# Autodesk Inventor assembly: Assembly_Opentrons_Autofocus_v1
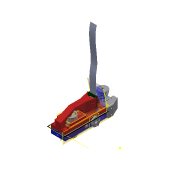
[picture p0: Inventor's stored thumbnail of the model, 180x180]
Saved by Autodesk Inventor 2019.4 (Build 234330000, 330)
## iProperties
Created: 2020-10-23
Part Number: Assembly_Opentrons_Autofocus_v1
Document SubType Name: Assembly
Designer: diederichbenedict
Author: diederichbenedict
## Documents named in this file (17)
- C:\Users\diederichbenedict\Dropbox\Dokumente\Promotion\PROJECTS\OPENTRONS\INVENTOR\Assembly_Opentrons_Autofocus_v1.iam
- C:\Users\diederichbenedict\Dropbox\Dokumente\Promotion\PROJECTS\OPENTRONS\INVENTOR\00_RasPi_Camera.ipt
- C:\Users\diederichbenedict\Dropbox\Dokumente\Promotion\PROJECTS\OPENTRONS\INVENTOR\00_IGUS_Drylin_RJ4JP-01-06.ipt
- C:\Users\diederichbenedict\Dropbox\Dokumente\Promotion\PROJECTS\OPENTRONS\INVENTOR\00_spindel_slide.ipt
- C:\Users\diederichbenedict\Dropbox\Dokumente\Promotion\PROJECTS\OPENTRONS\INVENTOR\00_objectivelens_10x.ipt
- C:\Users\diederichbenedict\Dropbox\Dokumente\Promotion\PROJECTS\OPENTRONS\INVENTOR\01_Slide_camera_x_v1.ipt
- C:\Users\diederichbenedict\Dropbox\Dokumente\Promotion\PROJECTS\OPENTRONS\INVENTOR\00_opticalpath.ipt
- C:\Users\diederichbenedict\Dropbox\Dokumente\Promotion\PROJECTS\OPENTRONS\INVENTOR\07_OPENTRONS_Autofocus_objectivemount_v0.ipt
- C:\Users\diederichbenedict\Dropbox\Dokumente\Promotion\PROJECTS\OPENTRONS\INVENTOR\00_COMAR_Mirror_10mm.ipt
- C:\Users\diederichbenedict\Dropbox\Dokumente\Promotion\PROJECTS\OPENTRONS\INVENTOR\08_Opentrons_Autofocus_flexurebaering.ipt
- C:\Users\diederichbenedict\Dropbox\Dokumente\Promotion\PROJECTS\OPENTRONS\INVENTOR\00_ESP32_Camera_only.ipt
- C:\Users\diederichbenedict\Dropbox\Dokumente\Promotion\PROJECTS\OPENTRONS\INVENTOR\00_Beampath_Autofocus _2.ipt
- C:\Users\diederichbenedict\Dropbox\Dokumente\Promotion\PROJECTS\OPENTRONS\INVENTOR\00_IR_Laserdiode.ipt
- C:\Users\diederichbenedict\Dropbox\Dokumente\Promotion\PROJECTS\OPENTRONS\INVENTOR\13_Opentrons_Autofocus_Objectivering_Laser_Cam.ipt
- C:\Users\diederichbenedict\Dropbox\Dokumente\Promotion\PROJECTS\OPENTRONS\INVENTOR\00_NEMA11.iam
- C:\Users\diederichbenedict\Dropbox\Dokumente\Promotion\PROJECTS\OPENTRONS\INVENTOR\OPENTRONS_Autofocus_NEMA_holder_tmp.ipt
- C:\Users\diederichbenedict\Dropbox\Dokumente\Promotion\PROJECTS\OPENTRONS\INVENTOR\OPENTRONS_Autofocus_spiral_Nema.ipt
## Components (16 placed, 16 different names)
1. 00_IGUS_Drylin_RJ4JP-01-06:1
2. 00_spindel_slide:1 — Insert:5
3. 01_Slide_camera_x_v1:1 — Insert:5, Mate:1, Mate:2, Flush:4, Angle:2, Flush:5, Flush:6, Angle:4, Flush:8, Flush:11, Mate:6, Mate:7, Flush:12, Flush:14, Flush:15
4. 00_objectivelens_10x:1 — Mate:1, Mate:2, Flush:2, Insert:10
5. 00_opticalpath:1 — Flush:4, Insert:7, Insert:8, Flush:9
6. 07_OPENTRONS_Autofocus_objectivemount_v0:1 — Flush:2
7. 00_COMAR_Mirror_10mm:1 — Insert:7
8. 00_RasPi_Camera:1 — Insert:8, Angle:2
9. 08_Opentrons_Autofocus_flexurebaering:1 — Flush:5, Flush:6
10. 00_ESP32_Camera_only:1 — Mate:4, Mate:5, Angle:5
11. 00_Beampath_Autofocus _2:1 — Insert:10, Mate:3, Mate:4, Angle:4
12. 00_IR_Laserdiode:1 — Mate:3, Flush:10
13. 13_Opentrons_Autofocus_Objectivering_Laser_Cam:1 — Flush:8, Flush:9, Flush:10, Flush:11, Mate:5, Angle:5
14. 00_NEMA11:1 [sub-assembly] — Mate:6, Mate:7, Flush:12, Insert:11
15. OPENTRONS_Autofocus_NEMA_holder_tmp:1 — Flush:14, Flush:15
16. OPENTRONS_Autofocus_spiral_Nema:1 — Insert:11
## Relationships (26: Flush 11, Mate 7, Insert 5, Angle 3)
- Insert:5: 00_spindel_slide:1 ↔ 01_Slide_camera_x_v1:1
- Mate:1: 01_Slide_camera_x_v1:1 ↔ 00_objectivelens_10x:1
- Mate:2 (17 mm): 01_Slide_camera_x_v1:1 ↔ 00_objectivelens_10x:1
- Flush:2: 00_objectivelens_10x:1 ↔ 07_OPENTRONS_Autofocus_objectivemount_v0:1
- Flush:4: 01_Slide_camera_x_v1:1 ↔ 00_opticalpath:1
- Insert:7: 00_opticalpath:1 ↔ 00_COMAR_Mirror_10mm:1
- Insert:8: 00_opticalpath:1 ↔ 00_RasPi_Camera:1
- Angle:2 (90 deg): 01_Slide_camera_x_v1:1 ↔ 00_RasPi_Camera:1
- Flush:5: 01_Slide_camera_x_v1:1 ↔ 08_Opentrons_Autofocus_flexurebaering:1
- Flush:6: 01_Slide_camera_x_v1:1 ↔ 08_Opentrons_Autofocus_flexurebaering:1
- Insert:10 (-2 mm): 00_objectivelens_10x:1 ↔ 00_Beampath_Autofocus _2:1
- Mate:3: 00_Beampath_Autofocus _2:1 ↔ 00_IR_Laserdiode:1
- Mate:4: 00_ESP32_Camera_only:1 ↔ 00_Beampath_Autofocus _2:1
- Angle:4 (145 deg): 01_Slide_camera_x_v1:1 ↔ 00_Beampath_Autofocus _2:1
- Flush:8: 01_Slide_camera_x_v1:1 ↔ 13_Opentrons_Autofocus_Objectivering_Laser_Cam:1
- Flush:9: 00_opticalpath:1 ↔ 13_Opentrons_Autofocus_Objectivering_Laser_Cam:1
- Flush:10: 00_IR_Laserdiode:1 ↔ 13_Opentrons_Autofocus_Objectivering_Laser_Cam:1
- Flush:11: 01_Slide_camera_x_v1:1 ↔ 13_Opentrons_Autofocus_Objectivering_Laser_Cam:1
- Mate:5: 00_ESP32_Camera_only:1 ↔ 13_Opentrons_Autofocus_Objectivering_Laser_Cam:1
- Angle:5 (0 deg): 00_ESP32_Camera_only:1 ↔ 13_Opentrons_Autofocus_Objectivering_Laser_Cam:1
- Mate:6 (0.25 mm): 01_Slide_camera_x_v1:1 ↔ 00_NEMA11:1
- Mate:7 (0.25 mm): 01_Slide_camera_x_v1:1 ↔ 00_NEMA11:1
- Flush:12: 01_Slide_camera_x_v1:1 ↔ 00_NEMA11:1
- Flush:14: 01_Slide_camera_x_v1:1 ↔ OPENTRONS_Autofocus_NEMA_holder_tmp:1
- Flush:15: 01_Slide_camera_x_v1:1 ↔ OPENTRONS_Autofocus_NEMA_holder_tmp:1
- Insert:11 (3 mm): 00_NEMA11:1 ↔ OPENTRONS_Autofocus_spiral_Nema:1
